# Autodesk Inventor assembly: CONTROLBOX2
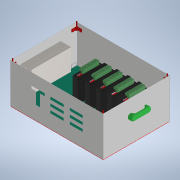
[picture p0: Inventor's stored thumbnail of the model, 180x180]
Saved by Autodesk Inventor 2020 (Build 240168000, 168)
## iProperties
Created: 2020-06-03
Part Number: CONTROLBOX2
Document SubType Name: Assembly
Designer: Gebruiker
Author: Gebruiker
## Documents named in this file (11)
- C:\Users\Gebruiker\Documents\GitHub\BeerMinder\3D-model\ControlBox\CONTROLBOX2.iam
- C:\Users\Gebruiker\Documents\GitHub\BeerMinder\3D-model\ControlBox\CONTROL_ONDERKANT.ipt
- C:\Users\Gebruiker\Documents\GitHub\BeerMinder\3D-model\ControlBox\CONTROL_LENGTE.ipt
- C:\Users\Gebruiker\Documents\GitHub\BeerMinder\3D-model\ControlBox\CONTROL_BREEDTE.ipt
- C:\Users\Gebruiker\Documents\GitHub\BeerMinder\3D-model\ControlBox\CONTOL_COMBI.ipt
- C:\Users\Gebruiker\Documents\GitHub\BeerMinder\3D-model\ControlBox\CONTROL_OPZETSTUK.ipt
- C:\Users\Gebruiker\Documents\GitHub\BeerMinder\3D-model\ControlBox\CONTROL_MONTEER.ipt
- C:\Users\Gebruiker\Documents\GitHub\BeerMinder\3D-model\ControlBox\controlbox_handvat.ipt
- C:\Users\Gebruiker\Documents\GitHub\BeerMinder\3D-model\ControlBox\ARDUINO DUE.iam
- C:\Users\Gebruiker\Documents\GitHub\BeerMinder\3D-model\ControlBox\Power supply unit.iam
- C:\Users\Gebruiker\Documents\GitHub\BeerMinder\3D-model\ControlBox\HY-DIV268N-5A.ipt
## Components (24 placed, 10 different names)
1. CONTROL_ONDERKANT:1 — Mate:1, Angle:1, Mate:2, Mate:3, Mate:6, Mate:10, Mate:11, Mate:14, Mate:17
2. CONTROL_LENGTE:1 — Mate:1, Angle:1, Mate:2, Mate:5, Mate:7, Mate:16, Mate:18, Mate:29, Mate:32
3. CONTROL_LENGTE:2 — Mate:3, Flush:1, Mate:9, Mate:13, Mate:25, Mate:28, Angle:6, Angle:7, Angle:8, Angle:9, Angle:10, Angle:11
4. CONTROL_BREEDTE:1 — Mate:5, Flush:1, Mate:12, Mate:19, Mate:27, Mate:30, Mate:34, Angle:3, Angle:5
5. CONTROL_BREEDTE:2 — Mate:6, Mate:7, Mate:8, Mate:15, Mate:26, Mate:31, Mate:33, Angle:2, Mate:36, Angle:4
6. CONTOL_COMBI:1 — Mate:17, Mate:18, Mate:19, Mate:20, Mate:23
7. CONTOL_COMBI:2 — Mate:11, Mate:12, Mate:13, Mate:21
8. CONTOL_COMBI:3 — Mate:14, Mate:15, Mate:16, Mate:22
9. CONTOL_COMBI:4 — Mate:8, Mate:9, Mate:10, Mate:24
10. CONTROL_OPZETSTUK:1 — Mate:20, Mate:21, Mate:22, Mate:23, Mate:24, Mate:35, Mate:37, Mate:38, Mate:39, Mate:40, Mate:41, Mate:42
11. CONTROL_MONTEER:1 — Mate:25, Mate:26
12. CONTROL_MONTEER:2 — Mate:27, Mate:28
13. CONTROL_MONTEER:3 — Mate:29, Mate:30
14. CONTROL_MONTEER:4 — Mate:31, Mate:32
15. controlbox_handvat:1 — Mate:34, Angle:3
16. controlbox_handvat:2 — Mate:33, Angle:2
17. ARDUINO DUE:1 [sub-assembly] — Mate:35, Angle:5
18. Power supply unit:1 [sub-assembly] — Mate:36, Angle:4
19. HY-DIV268N-5A:1 — Mate:37, Angle:6
20. HY-DIV268N-5A:2 — Mate:38, Angle:7
21. HY-DIV268N-5A:3 — Mate:39, Angle:8
22. HY-DIV268N-5A:4 — Mate:40, Angle:9
23. HY-DIV268N-5A:5 — Mate:41, Angle:10
24. HY-DIV268N-5A:6 — Mate:42, Angle:11
## Relationships (53: Mate 41, Angle 11, Flush 1)
- Mate:1: CONTROL_ONDERKANT:1 ↔ CONTROL_LENGTE:1
- Angle:1 (0 deg): CONTROL_ONDERKANT:1 ↔ CONTROL_LENGTE:1
- Mate:2: CONTROL_ONDERKANT:1 ↔ CONTROL_LENGTE:1
- Mate:3: CONTROL_ONDERKANT:1 ↔ CONTROL_LENGTE:2
- Mate:5: CONTROL_LENGTE:1 ↔ CONTROL_BREEDTE:1
- Flush:1: CONTROL_LENGTE:2 ↔ CONTROL_BREEDTE:1
- Mate:6: CONTROL_ONDERKANT:1 ↔ CONTROL_BREEDTE:2
- Mate:7: CONTROL_LENGTE:1 ↔ CONTROL_BREEDTE:2
- Mate:8: CONTROL_BREEDTE:2 ↔ CONTOL_COMBI:4
- Mate:9: CONTROL_LENGTE:2 ↔ CONTOL_COMBI:4
- Mate:10: CONTROL_ONDERKANT:1 ↔ CONTOL_COMBI:4
- Mate:11: CONTROL_ONDERKANT:1 ↔ CONTOL_COMBI:2
- Mate:12: CONTROL_BREEDTE:1 ↔ CONTOL_COMBI:2
- Mate:13: CONTROL_LENGTE:2 ↔ CONTOL_COMBI:2
- Mate:14: CONTROL_ONDERKANT:1 ↔ CONTOL_COMBI:3
- Mate:15: CONTROL_BREEDTE:2 ↔ CONTOL_COMBI:3
- Mate:16: CONTROL_LENGTE:1 ↔ CONTOL_COMBI:3
- Mate:17: CONTROL_ONDERKANT:1 ↔ CONTOL_COMBI:1
- Mate:18: CONTROL_LENGTE:1 ↔ CONTOL_COMBI:1
- Mate:19: CONTROL_BREEDTE:1 ↔ CONTOL_COMBI:1
- Mate:20: CONTOL_COMBI:1 ↔ CONTROL_OPZETSTUK:1
- Mate:21: CONTOL_COMBI:2 ↔ CONTROL_OPZETSTUK:1
- Mate:22: CONTOL_COMBI:3 ↔ CONTROL_OPZETSTUK:1
- Mate:23: CONTOL_COMBI:1 ↔ CONTROL_OPZETSTUK:1
- Mate:24: CONTOL_COMBI:4 ↔ CONTROL_OPZETSTUK:1
- Mate:25: CONTROL_LENGTE:2 ↔ CONTROL_MONTEER:1
- Mate:26: CONTROL_BREEDTE:2 ↔ CONTROL_MONTEER:1
- Mate:27: CONTROL_BREEDTE:1 ↔ CONTROL_MONTEER:2
- Mate:28: CONTROL_LENGTE:2 ↔ CONTROL_MONTEER:2
- Mate:29: CONTROL_LENGTE:1 ↔ CONTROL_MONTEER:3
- Mate:30: CONTROL_BREEDTE:1 ↔ CONTROL_MONTEER:3
- Mate:31: CONTROL_BREEDTE:2 ↔ CONTROL_MONTEER:4
- Mate:32: CONTROL_LENGTE:1 ↔ CONTROL_MONTEER:4
- Mate:33: CONTROL_BREEDTE:2 ↔ controlbox_handvat:2
- Angle:2 (0 deg): CONTROL_BREEDTE:2 ↔ controlbox_handvat:2
- Mate:34: CONTROL_BREEDTE:1 ↔ controlbox_handvat:1
- Angle:3 (0 deg): CONTROL_BREEDTE:1 ↔ controlbox_handvat:1
- Mate:35: CONTROL_OPZETSTUK:1 ↔ ARDUINO DUE:1
- Mate:36: CONTROL_BREEDTE:2 ↔ Power supply unit:1
- Angle:4 (0 deg): CONTROL_BREEDTE:2 ↔ Power supply unit:1
- Angle:5 (0 deg): CONTROL_BREEDTE:1 ↔ ARDUINO DUE:1
- Mate:37: CONTROL_OPZETSTUK:1 ↔ HY-DIV268N-5A:1
- Angle:6 (0 deg): CONTROL_LENGTE:2 ↔ HY-DIV268N-5A:1
- Mate:38: CONTROL_OPZETSTUK:1 ↔ HY-DIV268N-5A:2
- Angle:7 (0 deg): CONTROL_LENGTE:2 ↔ HY-DIV268N-5A:2
- Mate:39: CONTROL_OPZETSTUK:1 ↔ HY-DIV268N-5A:3
- Angle:8 (0 deg): CONTROL_LENGTE:2 ↔ HY-DIV268N-5A:3
- Mate:40: CONTROL_OPZETSTUK:1 ↔ HY-DIV268N-5A:4
- Angle:9 (0 deg): CONTROL_LENGTE:2 ↔ HY-DIV268N-5A:4
- Mate:41: CONTROL_OPZETSTUK:1 ↔ HY-DIV268N-5A:5
- Angle:10 (0 deg): CONTROL_LENGTE:2 ↔ HY-DIV268N-5A:5
- Mate:42: CONTROL_OPZETSTUK:1 ↔ HY-DIV268N-5A:6
- Angle:11 (0 deg): CONTROL_LENGTE:2 ↔ HY-DIV268N-5A:6
